# Autodesk Inventor assembly: 01
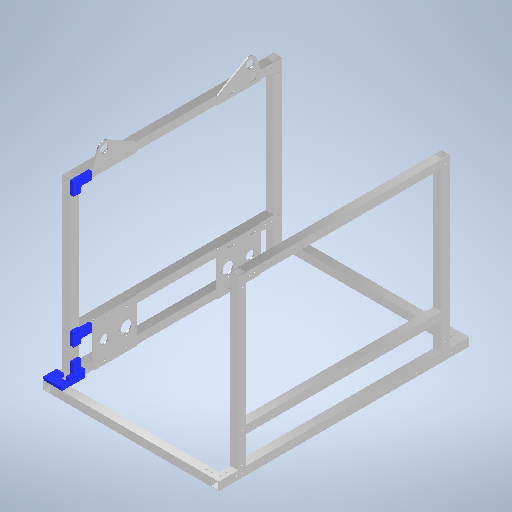
[picture p0: Inventor's stored thumbnail of the model, 512x512]
Saved by Autodesk Inventor 2025.1 (Build 291241000, 241)
## iProperties
Created: 2025-01-17
Part Number: 01
Document SubType Name: Assembly
Designer: yuki0520
Author: yuki0520
## Documents named in this file (9)
- C:\Users\yuki0520\OneDrive\ドキュメント\Inventor\2025_nhk\tanaka\motiage\01.iam
- C:\Users\yuki0520\OneDrive\ドキュメント\Inventor\2025_nhk\tanaka\motiage\ball_loading_v1_ASP_Base.ipt
- C:\Users\yuki0520\OneDrive\ドキュメント\Inventor\2025_nhk\tanaka\motiage\ball_loading_v1_Plate_left_down_M_F.ipt
- C:\Users\yuki0520\OneDrive\ドキュメント\Inventor\2025_nhk\tanaka\motiage\ball_loading_v1_Plate_left_up_F.ipt
- C:\Users\yuki0520\OneDrive\ドキュメント\Inventor\2025_nhk\tanaka\motiage\ball_loading_v1_Plate_right_down_M_F.ipt
- C:\Users\yuki0520\OneDrive\ドキュメント\Inventor\2025_nhk\tanaka\motiage\ball_loading_v1_Plate_up_F.ipt
- C:\Users\yuki0520\OneDrive\ドキュメント\Inventor\2025_nhk\tanaka\motiage\ball_loading_v1_Plate_ASP_F_1.ipt
- C:\Users\yuki0520\OneDrive\ドキュメント\Inventor\2025_nhk\tanaka\motiage\ball_loading_v1_Plate_ASP_F_2.ipt
- C:\Users\yuki0520\OneDrive\ドキュメント\Inventor\2025_nhk\tanaka\motiage\ball_loading_v1_Plate_ASP_F_3.ipt
## Components (9 placed, 8 different names)
1. ball_loading_v1_ASP_Base:1 — 挿入:1, 挿入:2, 挿入:3, 挿入:4, メイト:1, メイト:2, メイト:3, メイト:4, メイト:5, メイト:6, 挿入:5, 挿入:6, 挿入:7, 挿入:8, 挿入:9, 挿入:10, 挿入:11, 挿入:12, 挿入:13, 挿入:14, 挿入:15, 挿入:16, 挿入:17
2. ball_loading_v1_Plate_left_down_M_F:1 — 挿入:1, 挿入:2
3. ball_loading_v1_Plate_left_up_F:1 — 挿入:3, 挿入:4
4. ball_loading_v1_Plate_right_down_M_F:1 — メイト:1, メイト:2, メイト:3
5. ball_loading_v1_Plate_up_F:1 — メイト:4, メイト:5, メイト:6
6. ball_loading_v1_Plate_ASP_F_1:1 — 挿入:8, 挿入:9, 挿入:10
7. ball_loading_v1_Plate_ASP_F_2:1 — 挿入:5, 挿入:6, 挿入:7
8. ball_loading_v1_Plate_ASP_F_3:1 — 挿入:14, 挿入:15, 挿入:16, 挿入:17
9. ball_loading_v1_Plate_ASP_F_3:2 — 挿入:11, 挿入:12, 挿入:13
## Relationships (23: Insert 17, Mate 6)
- 挿入:1 [Insert]: ball_loading_v1_ASP_Base:1 ↔ ball_loading_v1_Plate_left_down_M_F:1
- 挿入:2 [Insert]: ball_loading_v1_ASP_Base:1 ↔ ball_loading_v1_Plate_left_down_M_F:1
- 挿入:3 [Insert]: ball_loading_v1_ASP_Base:1 ↔ ball_loading_v1_Plate_left_up_F:1
- 挿入:4 [Insert]: ball_loading_v1_ASP_Base:1 ↔ ball_loading_v1_Plate_left_up_F:1
- メイト:1 [Mate]: ball_loading_v1_ASP_Base:1 ↔ ball_loading_v1_Plate_right_down_M_F:1
- メイト:2 [Mate]: ball_loading_v1_ASP_Base:1 ↔ ball_loading_v1_Plate_right_down_M_F:1
- メイト:3 [Mate]: ball_loading_v1_ASP_Base:1 ↔ ball_loading_v1_Plate_right_down_M_F:1
- メイト:4 [Mate]: ball_loading_v1_ASP_Base:1 ↔ ball_loading_v1_Plate_up_F:1
- メイト:5 [Mate]: ball_loading_v1_ASP_Base:1 ↔ ball_loading_v1_Plate_up_F:1
- メイト:6 [Mate]: ball_loading_v1_ASP_Base:1 ↔ ball_loading_v1_Plate_up_F:1
- 挿入:5 [Insert]: ball_loading_v1_ASP_Base:1 ↔ ball_loading_v1_Plate_ASP_F_2:1
- 挿入:6 [Insert]: ball_loading_v1_ASP_Base:1 ↔ ball_loading_v1_Plate_ASP_F_2:1
- 挿入:7 [Insert]: ball_loading_v1_ASP_Base:1 ↔ ball_loading_v1_Plate_ASP_F_2:1
- 挿入:8 [Insert]: ball_loading_v1_ASP_Base:1 ↔ ball_loading_v1_Plate_ASP_F_1:1
- 挿入:9 [Insert]: ball_loading_v1_ASP_Base:1 ↔ ball_loading_v1_Plate_ASP_F_1:1
- 挿入:10 [Insert]: ball_loading_v1_ASP_Base:1 ↔ ball_loading_v1_Plate_ASP_F_1:1
- 挿入:11 [Insert]: ball_loading_v1_ASP_Base:1 ↔ ball_loading_v1_Plate_ASP_F_3:2
- 挿入:12 [Insert]: ball_loading_v1_ASP_Base:1 ↔ ball_loading_v1_Plate_ASP_F_3:2
- 挿入:13 [Insert]: ball_loading_v1_ASP_Base:1 ↔ ball_loading_v1_Plate_ASP_F_3:2
- 挿入:14 [Insert]: ball_loading_v1_ASP_Base:1 ↔ ball_loading_v1_Plate_ASP_F_3:1
- 挿入:15 [Insert]: ball_loading_v1_ASP_Base:1 ↔ ball_loading_v1_Plate_ASP_F_3:1
- 挿入:16 [Insert]: ball_loading_v1_ASP_Base:1 ↔ ball_loading_v1_Plate_ASP_F_3:1
- 挿入:17 [Insert]: ball_loading_v1_ASP_Base:1 ↔ ball_loading_v1_Plate_ASP_F_3:1
